# Autodesk Inventor assembly: Visual Assembly
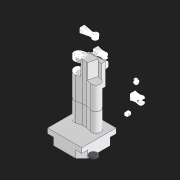
[picture p0: Inventor's stored thumbnail of the model, 180x180]
Saved by Autodesk Inventor 2017 SP1 (Build 210196100, 196)
## iProperties
Created: 2018-03-03
Part Number: Visual Assembly
Document SubType Name: Assembly
Designer: Zach
Author: Zach
## Documents named in this file (13)
- C:\Users\Zach\Documents\GitHub\tr1_description\meshes\Visual Assembly\Visual Assembly.iam
- C:\Users\Zach\Documents\GitHub\tr1_description\meshes\Visual Assembly\Base.ipt
- C:\Users\Zach\Documents\GitHub\tr1_description\meshes\Visual Assembly\Body.ipt
- C:\Users\Zach\Documents\GitHub\tr1_description\meshes\Visual Assembly\Wheel.ipt
- C:\Users\Zach\Documents\GitHub\tr1_description\meshes\Visual Assembly\Arm1.iam
- C:\Users\Zach\Documents\GitHub\tr1_description\meshes\Visual Assembly\Arm2.iam
- C:\Users\Zach\Documents\GitHub\tr1_description\meshes\Visual Assembly\Arm3.iam
- C:\Users\Zach\Documents\GitHub\tr1_description\meshes\Visual Assembly\Arm4.iam
- C:\Users\Zach\Documents\GitHub\tr1_description\meshes\Visual Assembly\Arm5.iam
- C:\Users\Zach\Documents\GitHub\tr1_description\meshes\Visual Assembly\Arm6.iam
- C:\Users\Zach\Documents\GitHub\tr1_description\meshes\Visual Assembly\Arm7.iam
- C:\Users\Zach\Documents\GitHub\tr1_description\meshes\Visual Assembly\Arm8.iam
- C:\Users\Zach\Documents\GitHub\tr1_description\meshes\Visual Assembly\Gripper1.iam
## Components (12 placed, 12 different names)
1. Base:1 — Mate:1, Mate:2, Mate:3
2. Body:1 — Mate:1, Mate:2, Mate:3, Mate:4, Mate:5, Mate:6
3. Wheel:1
4. Arm1:1 [sub-assembly] — Mate:4, Mate:5, Mate:6
5. Arm2:1 [sub-assembly]
6. Arm3:1 [sub-assembly]
7. Arm4:1 [sub-assembly]
8. Arm5:1 [sub-assembly]
9. Arm6:1 [sub-assembly]
10. Arm7:1 [sub-assembly]
11. Arm8:1 [sub-assembly]
12. Gripper1:1 [sub-assembly]
## Relationships (6: Mate 6)
- Mate:1: Base:1 ↔ Body:1
- Mate:2: Base:1 ↔ Body:1
- Mate:3: Base:1 ↔ Body:1
- Mate:4: Body:1 ↔ Arm1:1
- Mate:5: Body:1 ↔ Arm1:1
- Mate:6: Body:1 ↔ Arm1:1
